# Autodesk Inventor assembly: MotorPlate
Saved by Autodesk Inventor 2013 SP1 (Build 170176100, 176)
## iProperties
Created: 2013-12-02
Part Number: MotorPlate
Document SubType Name: Assembly
Designer: robotics
Author: robotics
## Documents named in this file (4)
- C:\Users\robotics\Documents\GitHub\2014-Preseason-Single-Speed-Gearbox\manufacture\assemblies\MotorPlate.iam
- C:\Users\robotics\Documents\GitHub\2014-Preseason-Single-Speed-Gearbox\manufacture\parts\Sheet Metal\GearboxPlate.ipt
- C:\Users\robotics\Documents\GitHub\2014-Preseason-Single-Speed-Gearbox\buy\VexPro\Bearings\217-2731-STEP\Imported Components\217-2731.20121205\217-2731.20121205.ipt
- C:\Users\robotics\Documents\GitHub\2014-Preseason-Single-Speed-Gearbox\buy\VexPro\Bearings\217-2733-STEP\Imported Components\217-2733.20121205\217-2733.20121205.ipt
## Components (3 placed, 3 different names)
1. GearboxPlate:1
2. 217-2731.20121205:1
3. 217-2733.20121205:1
## Relationships (4: Mate 4)
- [Mate]: GearboxPlate:1 ↔ 217-2731.20121205:1
- [Mate]: GearboxPlate:1 ↔ 217-2733.20121205:1
- [Mate]: GearboxPlate:1 ↔ 217-2733.20121205:1
- [Mate]: GearboxPlate:1 ↔ 217-2731.20121205:1
